# Autodesk Inventor assembly: BREEZE-S03
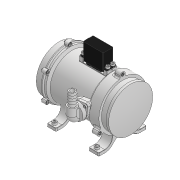
[picture p0: Inventor's stored thumbnail of the model, 180x180]
Saved by Autodesk Inventor 2020 (Build 240168000, 168)
## iProperties
Created: 2020-04-12
Part Number: BREEZE-S03
Description: AIR INLET ASSEMBLY
Document SubType Name: Assembly
Designer: John K
Author: John K
## Documents named in this file (15)
- C:\GrabCAD\MTL Ventilator Design\BREEZE\Subassemblies\BREEZE-S03.iam
- C:\GrabCAD\MTL Ventilator Design\BREEZE\Manufactured Parts\BREEZE-M11.ipt
- C:\GrabCAD\MTL Ventilator Design\BREEZE\Commercial Parts\McMaster\M5 Insert.ipt
- C:\GrabCAD\MTL Ventilator Design\BREEZE\Commercial Parts\McMaster\M4 Insert.ipt
- C:\GrabCAD\MTL Ventilator Design\BREEZE\Commercial Parts\McMaster\M3 Insert.ipt
- C:\GrabCAD\MTL Ventilator Design\BREEZE\Manufactured Parts\BREEZE-M13.ipt
- C:\GrabCAD\MTL Ventilator Design\BREEZE\Manufactured Parts\BREEZE-M14.ipt
- C:\GrabCAD\MTL Ventilator Design\BREEZE\Commercial Parts\Electronics\Servo Motor.ipt
- C:\GrabCAD\MTL Ventilator Design\BREEZE\Commercial Parts\Dust Filter.ipt
- C:\GrabCAD\MTL Ventilator Design\BREEZE\Commercial Parts\McMaster\M5x10mm Socket.ipt
- C:\GrabCAD\MTL Ventilator Design\BREEZE\Commercial Parts\McMaster\M4x8mm Socket.ipt
- C:\GrabCAD\MTL Ventilator Design\BREEZE\Commercial Parts\McMaster\M3x8mm Socket.ipt
- C:\GrabCAD\MTL Ventilator Design\BREEZE\Commercial Parts\McMaster\M3x6mm Nylon Screw.ipt
- C:\GrabCAD\MTL Ventilator Design\BREEZE\Commercial Parts\McMaster\O-Ring Dash 023.ipt
- C:\GrabCAD\MTL Ventilator Design\BREEZE\Manufactured Parts\BREEZE-M12.ipt
## Components (38 placed, 14 different names)
1. BREEZE-M11:1 — Insert:1, Mate:1, Insert:2, Insert:3, Insert:4, Insert:5, Insert:6, Insert:7, Insert:8, Insert:9, Insert:10, Insert:11, Insert:12, Mate:2, Tangent:1, Insert:13, Insert:14, Mate:5, Mate:7, Insert:24, Insert:25, Insert:26, Insert:27, Mate:8, Mate:9, Insert:35, Mate:11, Tangent:3
2. BREEZE-M12:1 — Insert:1, Mate:1, Insert:28, Insert:29
3. BREEZE-M13:1 — Insert:12
4. BREEZE-M14:1 — Mate:2, Tangent:1, Mate:3, Mate:4, Mate:6, Angle:1
5. Servo Motor:1 — Mate:5, Mate:6, Mate:7, Insert:30, Insert:31, Insert:32, Insert:33
6. Dust Filter:1 — Mate:8, Mate:9
7. O-Ring Dash 023:1 — Mate:11, Tangent:3
8. M3x8mm Socket:9
9. M3x6mm Nylon Screw:1 — Insert:35
10. M3x8mm Socket:1
11. M3x8mm Socket:2
12. M3x8mm Socket:3
13. M3x8mm Socket:4
14. M3x8mm Socket:5
15. M5x10mm Socket:1 — Insert:24
16. M5x10mm Socket:2 — Insert:25
17. M5x10mm Socket:3 — Insert:26
18. M5x10mm Socket:4 — Insert:27
19. M3x8mm Socket:6 — Insert:28
20. M3x8mm Socket:7 — Insert:29
21. M3x8mm Socket:8
22. M4x8mm Socket:1 — Insert:30
23. M4x8mm Socket:2 — Insert:31
24. M4x8mm Socket:3 — Insert:32
25. M4x8mm Socket:4 — Insert:33
26. M5 Insert:1 — Insert:2
27. M5 Insert:2 — Insert:3
28. M5 Insert:3 — Insert:4
29. M4 Insert:1 — Insert:5
30. M4 Insert:2 — Insert:6
31. M4 Insert:3 — Insert:7
32. M4 Insert:4 — Insert:8
33. M3 Insert:1 — Insert:9
34. M3 Insert:2 — Insert:10
35. M3 Insert:3 — Insert:11
36. M3 Insert:4 — Mate:3, Mate:4
37. M3 Insert:5 — Insert:14
38. M3 Insert:6 — Insert:13
## Relationships (46: Insert 31, Mate 12, Tangent 2, Angle 1)
- Insert:1: BREEZE-M11:1 ↔ BREEZE-M12:1
- Mate:1: BREEZE-M11:1 ↔ BREEZE-M12:1
- Insert:2: BREEZE-M11:1 ↔ M5 Insert:1
- Insert:3: BREEZE-M11:1 ↔ M5 Insert:2
- Insert:4: BREEZE-M11:1 ↔ M5 Insert:3
- Insert:5: BREEZE-M11:1 ↔ M4 Insert:1
- Insert:6: BREEZE-M11:1 ↔ M4 Insert:2
- Insert:7: BREEZE-M11:1 ↔ M4 Insert:3
- Insert:8: BREEZE-M11:1 ↔ M4 Insert:4
- Insert:9: BREEZE-M11:1 ↔ M3 Insert:1
- Insert:10: BREEZE-M11:1 ↔ M3 Insert:2
- Insert:11: BREEZE-M11:1 ↔ M3 Insert:3
- Insert:12: BREEZE-M11:1 ↔ BREEZE-M13:1
- Mate:2: BREEZE-M11:1 ↔ BREEZE-M14:1
- Tangent:1: BREEZE-M11:1 ↔ BREEZE-M14:1
- Mate:3: BREEZE-M14:1 ↔ M3 Insert:4
- Mate:4 (0.5 mm): BREEZE-M14:1 ↔ M3 Insert:4
- Insert:13: BREEZE-M11:1 ↔ M3 Insert:6
- Insert:14: BREEZE-M11:1 ↔ M3 Insert:5
- Mate:5: BREEZE-M11:1 ↔ Servo Motor:1
- Mate:6: BREEZE-M14:1 ↔ Servo Motor:1
- Mate:7: BREEZE-M11:1 ↔ Servo Motor:1
- Angle:1 (0 deg): BREEZE-M14:1
- [Insert]: BREEZE-M11:1 ↔ M3x8mm Socket:1
- [Insert]: BREEZE-M11:1 ↔ M3x8mm Socket:2
- [Insert]: BREEZE-M11:1 ↔ M3x8mm Socket:3
- [Insert]: BREEZE-M11:1 ↔ M3x8mm Socket:4
- [Insert]: BREEZE-M11:1 ↔ M3x8mm Socket:5
- Insert:24: BREEZE-M11:1 ↔ M5x10mm Socket:1
- Insert:25: BREEZE-M11:1 ↔ M5x10mm Socket:2
- Insert:26: BREEZE-M11:1 ↔ M5x10mm Socket:3
- Insert:27: BREEZE-M11:1 ↔ M5x10mm Socket:4
- Insert:28: BREEZE-M12:1 ↔ M3x8mm Socket:6
- Insert:29: BREEZE-M12:1 ↔ M3x8mm Socket:7
- Insert:30: Servo Motor:1 ↔ M4x8mm Socket:1
- Insert:31: Servo Motor:1 ↔ M4x8mm Socket:2
- Insert:32: Servo Motor:1 ↔ M4x8mm Socket:3
- Insert:33: Servo Motor:1 ↔ M4x8mm Socket:4
- [Insert]: BREEZE-M11:1 ↔ M3x8mm Socket:8
- Mate:8: BREEZE-M11:1 ↔ Dust Filter:1
- Mate:9: BREEZE-M11:1 ↔ Dust Filter:1
- [Mate]: BREEZE-M11:1 ↔ M3x8mm Socket:9
- Insert:35: BREEZE-M11:1 ↔ M3x6mm Nylon Screw:1
- Mate:11: BREEZE-M11:1 ↔ O-Ring Dash 023:1
- Tangent:3: BREEZE-M11:1 ↔ O-Ring Dash 023:1
- [Mate]: BREEZE-M11:1 ↔ M3x8mm Socket:9
